# Autodesk Inventor assembly: MG_996R
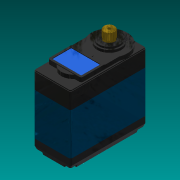
[picture p0: Inventor's stored thumbnail of the model, 180x180]
Saved by Autodesk Inventor 2020.3 (Build 243373000, 373)
## iProperties
Created: 2016-09-26
Part Number: MG_996R
Document SubType Name: Assembly
Designer: Julian
Author: Julian
## Documents named in this file (5)
- C:\Users\Svend\OneDrive\Documents\GitHub\BeerMinder\3D-model\servo\MG_996R.iam
- C:\Users\Svend\OneDrive\Documents\GitHub\BeerMinder\3D-model\servo\Base.ipt
- C:\Users\Svend\OneDrive\Documents\GitHub\BeerMinder\3D-model\servo\Medio.ipt
- C:\Users\Svend\OneDrive\Documents\GitHub\BeerMinder\3D-model\servo\Top.ipt
- C:\Users\Svend\OneDrive\Documents\GitHub\BeerMinder\3D-model\servo\Eje.ipt
## Components (4 placed, 4 different names)
1. Top:1 — Mate:1, Mate:2, Flush:1, Flush:2, Flush:3
2. Medio:1 — Rígido:1, Angle:1, Mate:2, Flush:1, Flush:2
3. Base:1 — Rígido:1
4. Eje:1 — Angle:1, Mate:1, Flush:3
## Relationships (7: Flush 3, Mate 2, WeldJoint 1, Angle 1)
- Rígido:1 [WeldJoint]: Medio:1 ↔ Base:1
- Angle:1 (0 deg): Medio:1 ↔ Eje:1
- Mate:1: Top:1 ↔ Eje:1
- Mate:2: Top:1 ↔ Medio:1
- Flush:1: Top:1 ↔ Medio:1
- Flush:2: Top:1 ↔ Medio:1
- Flush:3 (-4.5 mm): Top:1 ↔ Eje:1
